# Autodesk Inventor assembly: templete_t265cover
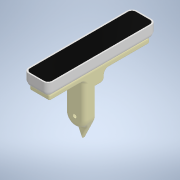
[picture p0: Inventor's stored thumbnail of the model, 180x180]
Saved by Autodesk Inventor 2022 (Build 260153000, 153)
## iProperties
Created: 2021-12-10
Part Number: templete_t265cover
Document SubType Name: Assembly
Designer: ARRF
Author: ARRF
## Documents named in this file (3)
- C:\Users\ARRF\My Drive (sasa.kuruppuarachchi@gmail.com)\KNU\ARRF\XR project\jetson_cv_hub_ver1\templete_t265cover.iam
- C:\Users\ARRF\My Drive (sasa.kuruppuarachchi@gmail.com)\KNU\ARRF\XR project\jetson_cv_hub_ver1\t265_mount_imm_secondary.ipt
- C:\Users\ARRF\My Drive (sasa.kuruppuarachchi@gmail.com)\KNU\ARRF\XR project\jetson_cv_hub_ver1\External_models\t265ass_Simplify_1.ipt
## Components (2 placed, 2 different names)
1. t265_mount_imm_secondary:1 — Mate:1, Mate:2, Mate:3
2. t265ass_Simplify_1:1 — Mate:1, Mate:2, Mate:3
## Relationships (3: Mate 3)
- Mate:1: t265_mount_imm_secondary:1 ↔ t265ass_Simplify_1:1
- Mate:2: t265_mount_imm_secondary:1 ↔ t265ass_Simplify_1:1
- Mate:3: t265_mount_imm_secondary:1 ↔ t265ass_Simplify_1:1
